# Autodesk Inventor assembly: Arduino Nano - Soldered
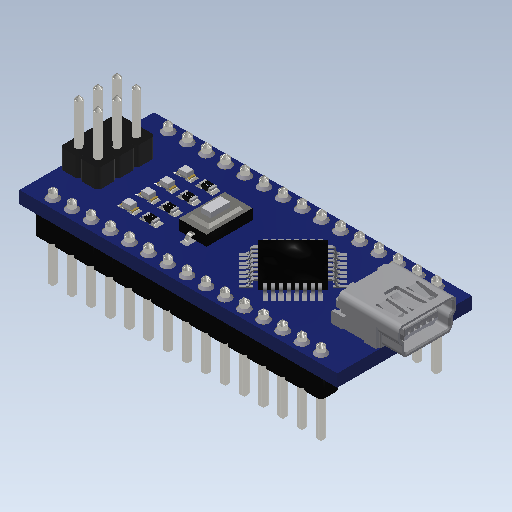
[picture p0: Inventor's stored thumbnail of the model, 512x512]
Saved by Autodesk Inventor 2020 (Build 240168000, 168)
## iProperties
Created: 2017-10-26
Part Number: Arduino Nano - Soldered
Document SubType Name: Weldment
Designer: Alex
Weld Material: Welded Aluminum-6061
Author: Alex
## Documents named in this file (9)
- C:\Users\amsmi\Google Drive\Pirani Gauge\Pirani Gauge Modeling\Data Acquisition\Arduino Nano - Soldered.iam
- C:\Users\amsmi\Google Drive\Pirani Gauge\Pirani Gauge Modeling\Data Acquisition\Arduino Nano.ipt
- C:\Users\amsmi\Google Drive\Pirani Gauge\Pirani Gauge Modeling\Data Acquisition\USB-Mini-B.ipt
- C:\Users\amsmi\Google Drive\Pirani Gauge\Pirani Gauge Modeling\Data Acquisition\2x3 header.ipt
- C:\Users\amsmi\Google Drive\Pirani Gauge\Pirani Gauge Modeling\Data Acquisition\15 pin header - round.ipt
- C:\Users\amsmi\Google Drive\Pirani Gauge\Pirani Gauge Modeling\Data Acquisition\TO-243AA.ipt
- C:\Users\amsmi\Google Drive\Pirani Gauge\Pirani Gauge Modeling\Data Acquisition\Switch.ipt
- C:\Users\amsmi\Google Drive\Pirani Gauge\Pirani Gauge Modeling\Data Acquisition\Black 0603 - Soldered.ipt
- C:\Users\amsmi\Google Drive\Pirani Gauge\Pirani Gauge Modeling\Data Acquisition\LED-0603H0.75 - Soldered.ipt
## Components (15 placed, 8 different names)
1. Arduino Nano:1 — Mate:1, Mate:2, Mate:3, Mate:5, Flush:2, Mate:7, Mate:8, Mate:9, Mate:12, Mate:13, Mate:14, Mate:15, Mate:16, Mate:17, Flush:3, Flush:4, Mate:19, Angle:1, Flush:5, Flush:6, Mate:22, Angle:2, Flush:24, Flush:25, Mate:23, Mate:24
2. USB-Mini-B:1 — Mate:5, Flush:2
3. 2x3 header:1 — Mate:7, Mate:8, Mate:9
4. 15 pin header - round:1 — Mate:14, Mate:15, Mate:17
5. 15 pin header - round:2 — Mate:12, Mate:13, Mate:16
6. TO-243AA:1 — Mate:19, Angle:1, Flush:5, Flush:6
7. Switch:1 — Mate:22, Angle:2, Flush:24, Flush:25
8. Black 0603 - Soldered:1 — Flush:3, Flush:4, Mate:23, Flush:26, Mate:25
9. LED-0603H0.75 - Soldered:1 — Mate:24, Flush:26, Mate:25
10. Black 0603 - Soldered:2
11. LED-0603H0.75 - Soldered:2
12. Black 0603 - Soldered:3
13. LED-0603H0.75 - Soldered:3
14. Black 0603 - Soldered:4
15. LED-0603H0.75 - Soldered:4
## Component patterns: (4 elements, first: Black 0603 - Soldered:1 + LED-0603H0.75 - Soldered:1)
## Relationships (28: Mate 18, Flush 8, Angle 2)
- Mate:1: Arduino Nano:1
- Mate:2: Arduino Nano:1
- Mate:3: Arduino Nano:1
- Mate:5: Arduino Nano:1 ↔ USB-Mini-B:1
- Flush:2: Arduino Nano:1 ↔ USB-Mini-B:1
- Mate:7: Arduino Nano:1 ↔ 2x3 header:1
- Mate:8: Arduino Nano:1 ↔ 2x3 header:1
- Mate:9: Arduino Nano:1 ↔ 2x3 header:1
- Mate:12: Arduino Nano:1 ↔ 15 pin header - round:2
- Mate:13: Arduino Nano:1 ↔ 15 pin header - round:2
- Mate:14: Arduino Nano:1 ↔ 15 pin header - round:1
- Mate:15: Arduino Nano:1 ↔ 15 pin header - round:1
- Mate:16: Arduino Nano:1 ↔ 15 pin header - round:2
- Mate:17: Arduino Nano:1 ↔ 15 pin header - round:1
- Flush:3 (-4.75 mm): Arduino Nano:1 ↔ Black 0603 - Soldered:1
- Flush:4 (11.5 mm): Arduino Nano:1 ↔ Black 0603 - Soldered:1
- Mate:19: Arduino Nano:1 ↔ TO-243AA:1
- Angle:1 (0 deg): Arduino Nano:1 ↔ TO-243AA:1
- Flush:5 (5.9 mm): Arduino Nano:1 ↔ TO-243AA:1
- Flush:6 (3.683 mm): Arduino Nano:1 ↔ TO-243AA:1
- Mate:22: Arduino Nano:1 ↔ Switch:1
- Angle:2 (0 deg): Arduino Nano:1 ↔ Switch:1
- Flush:24: Arduino Nano:1 ↔ Switch:1
- Flush:25 (15.24 mm): Arduino Nano:1 ↔ Switch:1
- Mate:23: Arduino Nano:1 ↔ Black 0603 - Soldered:1
- Mate:24: Arduino Nano:1 ↔ LED-0603H0.75 - Soldered:1
- Flush:26 (0.0508 mm): Black 0603 - Soldered:1 ↔ LED-0603H0.75 - Soldered:1
- Mate:25 (1.27 mm): Black 0603 - Soldered:1 ↔ LED-0603H0.75 - Soldered:1
